# Autodesk Inventor assembly: Square Frame
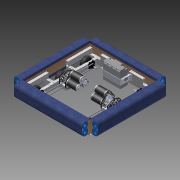
[picture p0: Inventor's stored thumbnail of the model, 180x180]
Saved by Autodesk Inventor 2015 SP1 (Build 190203100, 203)
## iProperties
Created: 2014-12-21
Part Number: Square Frame
Document SubType Name: Assembly
Designer: Jarod
Author: Jarod
## Documents named in this file (23)
- C:\Users\Jarod\Documents\Westview\Robotics\FRC\2015\CAD\Ideas\Square Frame\Square Frame.iam
- C:\Users\Jarod\Documents\Westview\Robotics\FRC\2015\CAD\Ideas\Square Frame\Square Frame Parts\frame_wide.ipt
- C:\Users\Jarod\Documents\Westview\Robotics\FRC\2015\CAD\Ideas\Square Frame\Square Frame Parts\frame_long.ipt
- C:\Users\Jarod\Documents\Westview\Robotics\FRC\2015\CAD\Ideas\Square Frame\Square Frame Parts\Imported Components\Versablock (217-3432)\Versablock (217-3432).ipt
- C:\Users\Jarod\Documents\Westview\Robotics\FRC\2015\CAD\Ideas\Square Frame\Square Frame Parts\Imported Components\0.5 hex bearing (217-2734)\0.5 hex bearing (217-2734).ipt
- C:\Users\Jarod\Documents\Westview\Robotics\FRC\2015\CAD\Ideas\Square Frame\Square Frame Parts\Imported Components\VersaFrame Gusset (217-3557)\VersaFrame Gusset (217-3557).ipt
- C:\Users\Jarod\Documents\Westview\Robotics\FRC\2015\CAD\Ideas\Square Frame\Square Frame Parts\Imported Components\Colson Wheel (4 x 1.5, 0.5 Hex bore) (217-4052)\Colson Wheel (4 x 1.5, 0.5 Hex bore) (217-4052).ipt
- C:\Users\Jarod\Documents\Westview\Robotics\FRC\2015\CAD\Ideas\Square Frame\Square Frame Parts\Imported Components\WCP Single Speed, Double Reduction Gearbox, West Coast Version (217-3422)\WCP Single Speed, Doub.iam
- C:\Users\Jarod\Documents\Westview\Robotics\FRC\2015\CAD\Ideas\Square Frame\Square Frame Parts\Imported Components\0.5 hex hub #35 sprocket 15t double (217-2656)\0.5 hex hub #35 sprocket 15t double (217-2656).ipt
- C:\Users\Jarod\Documents\Westview\Robotics\FRC\2015\CAD\Ideas\Square Frame\Square Frame Parts\Imported Components\0.5 hex hub #35 sprocket 15t (217-2660)\0.5 hex hub #35 sprocket 15t (217-2660).ipt
- C:\Users\Jarod\Documents\Westview\Robotics\FRC\2015\CAD\Ideas\Square Frame\Square Frame Parts\axle.ipt
- C:\Users\Jarod\Documents\Westview\Robotics\FRC\2015\CAD\Ideas\Square Frame\Square Frame Parts\Imported Components\0.5 hex collar (217-2737)\0.5 hex collar (217-2737).ipt
- C:\Users\Jarod\Documents\Westview\Robotics\FRC\2015\CAD\Ideas\Square Frame\Square Frame Parts\Imported Components\WCP Single Speed, Double Reduction Gearbox, West Coast Version (217-3422)\217-2758-001 Rev1.ipt
- C:\Users\Jarod\Documents\Westview\Robotics\FRC\2015\CAD\Ideas\Square Frame\Square Frame Parts\Imported Components\WCP Cam (217-3431)\WCP Cam (217-3431).ipt
- C:\Users\Jarod\Documents\Westview\Robotics\FRC\2015\CAD\Ideas\Square Frame\Square Frame Parts\base.ipt
- C:\Users\Jarod\Documents\Westview\Robotics\FRC\2015\CAD\Ideas\Square Frame\Square Frame Parts\frame_side.ipt
- C:\Users\Jarod\Documents\Westview\Robotics\FRC\2015\CAD\Ideas\Square Frame\Square Frame Parts\frame_side_bumper.ipt
- C:\Users\Jarod\Documents\Westview\Robotics\FRC\2015\CAD\Ideas\Square Frame\Square Frame Parts\bumper.iam
- C:\Users\Jarod\Documents\Westview\Robotics\FRC\2015\CAD\Ideas\Square Frame\Square Frame Parts\frame_front_bumper.ipt
- C:\Users\Jarod\Documents\Westview\Robotics\FRC\2015\CAD\Ideas\Square Frame\Square Frame Parts\chain (71 links).ipt
- C:\Users\Jarod\Documents\Westview\Robotics\FRC\2015\CAD\Ideas\Square Frame\Square Frame Parts\Imported Components\VersaFrame Gusset (217-3557)\VersaFrame Gusset (217-3557) (modified).ipt
- C:\Users\Jarod\Documents\Westview\Robotics\FRC\2015\CAD\Ideas\Square Frame\Square Frame Parts\battery.ipt
- C:\Users\Jarod\Documents\Westview\Robotics\FRC\2015\CAD\Ideas\Square Frame\Square Frame Parts\Imported Components\Battery Tray\Battery Tray_TOP.iam
## Components (95 placed, 22 different names)
1. frame_wide:1 — Flush:1, Flush:2, Flush:3, Mate:1, Mate:2, Mate:28, Mate:29, Mate:38, Mate:39, Mate:52, Mate:53, Flush:13, Flush:14, Mate:56, Mate:57, Flush:23, Flush:24, Flush:37, Flush:63, Flush:64, Mate:186, Flush:65, Flush:66, Mate:188, Flush:69, Flush:70, Mate:190, Flush:75, Flush:76, Mate:192, Mate:194, Flush:77, Mate:198, Flush:79, Mate:204, Flush:82, Mate:235, Mate:236
2. frame_wide:2 — Flush:3, Mate:3, Mate:32, Mate:33, Mate:34, Mate:35, Mate:54, Mate:55, Flush:17, Flush:18, Mate:58, Mate:59, Flush:25, Flush:26, Flush:63, Mate:187, Mate:189, Flush:71, Flush:72, Flush:73, Flush:74, Mate:195, Flush:78, Mate:200, Flush:80, Mate:202, Flush:81, Mate:232, Mate:233, Mate:234, Mate:237, Mate:238
3. frame_long:1 — Flush:1, Mate:2, Mate:3, Mate:4, Mate:5, Mate:8, Mate:9, Mate:16, Mate:17, Mate:20, Mate:21, Flush:15, Flush:16, Flush:19, Flush:20, Mate:60, Mate:61, Mate:64, Mate:65, Mate:72, Mate:73, Mate:74, Mate:161, Mate:162, Cylindrical:15, Cylindrical:16, Flush:38, Flush:39, Flush:40, Mate:166, Mate:167, Mate:181, Flush:64, Mate:208, Mate:209, Mate:210, Mate:211, Mate:220, Flush:83, Mate:221, Flush:84, Mate:222, Flush:85, Mate:223, Flush:86, Mate:228, Mate:229
4. frame_long:2 — Flush:2, Mate:1, Mate:10, Mate:11, Mate:14, Mate:15, Mate:22, Mate:23, Mate:26, Mate:27, Flush:21, Flush:22, Flush:27, Flush:28, Mate:66, Mate:67, Mate:70, Mate:71, Mate:75, Mate:76, Mate:77, Mate:159, Mate:160, Cylindrical:13, Cylindrical:14, Flush:41, Flush:42, Mate:181, Mate:184, Mate:185, Mate:212, Mate:213, Mate:214, Mate:215, Mate:224, Flush:87, Mate:225, Flush:88, Mate:226, Flush:89, Mate:227, Flush:90, Mate:230, Mate:231
5. frame_side:1 — Flush:39, Mate:166, Flush:91, Flush:92
6. frame_side:2 — Flush:40, Mate:167, Flush:93, Flush:94
7. frame_side:3 — Flush:41, Mate:184, Flush:95, Flush:96
8. frame_side:4 — Flush:42, Mate:185, Flush:97, Flush:98
9. frame_side_bumper:1 — Mate:186, Flush:65, Flush:66, Mate:196
10. frame_side_bumper:2 — Mate:187, Flush:71, Flush:72
11. frame_side_bumper:3 — Mate:188, Flush:69, Flush:70, Mate:197
12. frame_side_bumper:4 — Mate:189, Flush:73, Flush:74
13. frame_front_bumper:1 — Mate:198, Flush:79, Mate:236, Mate:239
14. frame_front_bumper:2 — Mate:200, Flush:80, Mate:238, Mate:240
15. frame_front_bumper:3 — Mate:204, Flush:82, Mate:235
16. frame_front_bumper:4 — Mate:202, Flush:81, Mate:237
17. base:1 — Mate:163, Flush:37, Flush:38
18. VersaFrame Gusset (217-3557):1 — Mate:52, Flush:13, Flush:15
19. VersaFrame Gusset (217-3557):2 — Mate:53, Flush:14, Flush:16, Mate:163
20. VersaFrame Gusset (217-3557):3 — Mate:54, Flush:17, Flush:20
21. VersaFrame Gusset (217-3557):4 — Mate:55, Flush:18, Flush:19
22. VersaFrame Gusset (217-3557):5 — Mate:57, Flush:22, Flush:23
23. VersaFrame Gusset (217-3557):6 — Mate:56, Flush:21, Flush:24
24. VersaFrame Gusset (217-3557):7 — Mate:58, Flush:25, Flush:28
25. VersaFrame Gusset (217-3557):8 — Mate:59, Flush:26, Flush:27
26. VersaFrame Gusset (217-3557) (modified):1 — Mate:220, Flush:83, Flush:91, Mate:228
27. VersaFrame Gusset (217-3557) (modified):2 — Mate:221, Flush:84, Flush:92
28. VersaFrame Gusset (217-3557) (modified):3 — Mate:222, Flush:85, Flush:93, Mate:229
29. VersaFrame Gusset (217-3557) (modified):4 — Mate:223, Flush:86, Flush:94
30. VersaFrame Gusset (217-3557) (modified):5 — Mate:224, Flush:87, Flush:95, Mate:230
31. VersaFrame Gusset (217-3557) (modified):6 — Mate:225, Flush:88, Flush:96
32. VersaFrame Gusset (217-3557) (modified):7 — Mate:226, Flush:89, Flush:97, Mate:231
33. VersaFrame Gusset (217-3557) (modified):8 — Mate:227, Flush:90, Flush:98
34. bumper:1 [sub-assembly] — Mate:190, Flush:75, Mate:196
35. bumper:2 [sub-assembly] — Flush:76, Mate:192, Mate:197
36. bumper:3 [sub-assembly] — Mate:194, Flush:77, Mate:239
37. bumper:4 [sub-assembly] — Mate:195, Flush:78, Mate:240
38. WCP Single Speed, Doub:1 [sub-assembly] — Mate:72, Mate:73, Mate:74, Mate:81, Mate:82, Mate:83, Mate:90, Mate:91, Mate:128, Mate:129, Mate:130
39. WCP Single Speed, Doub:2 [sub-assembly] — Mate:75, Mate:76, Mate:77, Mate:78, Mate:79, Mate:80, Mate:104, Mate:105, Mate:148, Mate:149, Mate:150
40. Versablock (217-3432):1 — Mate:4, Mate:17, Mate:38, Cylindrical:2
41. Versablock (217-3432):2 — Mate:5, Mate:16, Mate:39, Cylindrical:1
42. Versablock (217-3432):5 — Mate:9, Mate:21, Mate:34, Cylindrical:5
43. Versablock (217-3432):6 — Mate:8, Mate:20, Mate:35, Cylindrical:6
44. Versablock (217-3432):7 — Mate:10, Mate:22, Mate:28, Cylindrical:7
45. Versablock (217-3432):8 — Mate:11, Mate:23, Mate:29, Cylindrical:8
46. Versablock (217-3432):11 — Mate:14, Mate:27, Mate:32, Cylindrical:11
47. Versablock (217-3432):12 — Mate:15, Mate:26, Mate:33, Cylindrical:12
48. axle:1 — Mate:84, Mate:85, Mate:86, Mate:87, Mate:88, Mate:89, Mate:118, Mate:119, Mate:120, Mate:121, Mate:122, Mate:123, Flush:33
49. axle:2 — Mate:92, Mate:93, Mate:94, Mate:95, Mate:96, Mate:97, Mate:114, Mate:115, Mate:132, Mate:133, Mate:134, Mate:135, Flush:34
50. axle:3 — Mate:98, Mate:99, Mate:100, Mate:101, Mate:102, Mate:103, Mate:138, Mate:139, Mate:140, Mate:141, Mate:142, Mate:143, Flush:35
51. axle:4 — Mate:106, Mate:107, Mate:108, Mate:109, Mate:110, Mate:111, Mate:112, Mate:113, Mate:152, Mate:153, Mate:156, Mate:157, Flush:36
52. 0.5 hex bearing (217-2734):1 — Mate:60, Cylindrical:1, Mate:88, Mate:89, Mate:126
53. 0.5 hex bearing (217-2734):2 — Mate:61, Cylindrical:2
54. 0.5 hex bearing (217-2734):5 — Mate:64, Cylindrical:6, Mate:96, Mate:97, Mate:180
55. 0.5 hex bearing (217-2734):6 — Mate:65, Cylindrical:5, Mate:116
56. 0.5 hex bearing (217-2734):7 — Mate:66, Cylindrical:8, Mate:102, Mate:103, Mate:146
57. 0.5 hex bearing (217-2734):8 — Mate:67, Cylindrical:7
58. 0.5 hex bearing (217-2734):11 — Mate:70, Cylindrical:12, Mate:110, Mate:111, Mate:155
59. 0.5 hex bearing (217-2734):12 — Mate:71, Cylindrical:11, Mate:117
60. Colson Wheel (4 x 1.5, 0.5 Hex bore) (217-4052):2 — Mate:90, Mate:91, Mate:128, Mate:131
61. Colson Wheel (4 x 1.5, 0.5 Hex bore) (217-4052):3 — Mate:92, Mate:93, Mate:136, Mate:180
62. Colson Wheel (4 x 1.5, 0.5 Hex bore) (217-4052):4 — Mate:98, Mate:99, Mate:146, Mate:147
63. Colson Wheel (4 x 1.5, 0.5 Hex bore) (217-4052):5 — Mate:104, Mate:105, Mate:148, Mate:151
64. Colson Wheel (4 x 1.5, 0.5 Hex bore) (217-4052):6 — Mate:106, Mate:107, Mate:155, Mate:158
65. Colson Wheel (4 x 1.5, 0.5 Hex bore) (217-4052):1 — Mate:84, Mate:85, Mate:126, Mate:127
66. 0.5 hex hub #35 sprocket 15t double (217-2656):1 — Mate:78, Mate:79, Mate:80, Flush:31, Flush:32
67. 0.5 hex hub #35 sprocket 15t double (217-2656):2 — Mate:81, Mate:82, Mate:83, Flush:29, Flush:30
68. 0.5 hex hub #35 sprocket 15t (217-2660):1 — Flush:32, Mate:108, Mate:109, Mate:154, Mate:217
69. 0.5 hex hub #35 sprocket 15t (217-2660):2 — Flush:29, Mate:94, Mate:95, Mate:137, Mate:218
70. 0.5 hex hub #35 sprocket 15t (217-2660):3 — Flush:30, Mate:86, Mate:87, Mate:124, Mate:125, Mate:219
71. 0.5 hex hub #35 sprocket 15t (217-2660):4 — Flush:31, Mate:100, Mate:101, Mate:144, Mate:145, Mate:216
72. 217-2758-001 Rev1:1 — Mate:112, Mate:113, Mate:117
73. 217-2758-001 Rev1:2 — Mate:114, Mate:115, Mate:116
74. 0.5 hex collar (217-2737):1 — Mate:118, Mate:119, Mate:127, Flush:33
75. 0.5 hex collar (217-2737):2 — Mate:120, Mate:121, Mate:125
76. 0.5 hex collar (217-2737):3 — Mate:122, Mate:123, Mate:124
77. 0.5 hex collar (217-2737):4 — Mate:129, Mate:130, Mate:131
78. 0.5 hex collar (217-2737):5 — Mate:134, Mate:135, Mate:136, Flush:34
79. 0.5 hex collar (217-2737):6 — Mate:132, Mate:133, Mate:137
80. 0.5 hex collar (217-2737):7 — Mate:142, Mate:143, Mate:147, Flush:35
81. 0.5 hex collar (217-2737):8 — Mate:140, Mate:141, Mate:145
82. 0.5 hex collar (217-2737):9 — Mate:138, Mate:139, Mate:144
83. 0.5 hex collar (217-2737):10 — Mate:149, Mate:150, Mate:151
84. 0.5 hex collar (217-2737):11 — Mate:156, Mate:157, Mate:158, Flush:36
85. 0.5 hex collar (217-2737):12 — Mate:152, Mate:153, Mate:154
86. chain (71 links):1 — Mate:208, Mate:209, Mate:219
87. chain (71 links):2 — Mate:210, Mate:211, Mate:218
88. chain (71 links):3 — Mate:212, Mate:213, Mate:216
89. chain (71 links):4 — Mate:214, Mate:215, Mate:217
90. WCP Cam (217-3431):1 — Mate:162, Cylindrical:16
91. WCP Cam (217-3431):2 — Mate:161, Cylindrical:15
92. WCP Cam (217-3431):3 — Mate:160, Cylindrical:14
93. WCP Cam (217-3431):4 — Mate:159, Cylindrical:13
94. battery:1
95. Battery Tray_TOP:1 [sub-assembly] — Mate:232, Mate:233, Mate:234
## Relationships (267: Mate 188, Flush 67, CylindricalJoint 12)
- Flush:1: frame_wide:1 ↔ frame_long:1
- Flush:2: frame_wide:1 ↔ frame_long:2
- Flush:3: frame_wide:1 ↔ frame_wide:2
- Mate:1: frame_wide:1 ↔ frame_long:2
- Mate:2: frame_wide:1 ↔ frame_long:1
- Mate:3: frame_wide:2 ↔ frame_long:1
- Mate:4: frame_long:1 ↔ Versablock (217-3432):1
- Mate:5: frame_long:1 ↔ Versablock (217-3432):2
- Mate:8: frame_long:1 ↔ Versablock (217-3432):6
- Mate:9: frame_long:1 ↔ Versablock (217-3432):5
- Mate:10: frame_long:2 ↔ Versablock (217-3432):7
- Mate:11: frame_long:2 ↔ Versablock (217-3432):8
- Mate:14: frame_long:2 ↔ Versablock (217-3432):11
- Mate:15: frame_long:2 ↔ Versablock (217-3432):12
- Mate:16: frame_long:1 ↔ Versablock (217-3432):2
- Mate:17: frame_long:1 ↔ Versablock (217-3432):1
- Mate:20: frame_long:1 ↔ Versablock (217-3432):6
- Mate:21: frame_long:1 ↔ Versablock (217-3432):5
- Mate:22: frame_long:2 ↔ Versablock (217-3432):7
- Mate:23: frame_long:2 ↔ Versablock (217-3432):8
- Mate:26: frame_long:2 ↔ Versablock (217-3432):12
- Mate:27: frame_long:2 ↔ Versablock (217-3432):11
- Mate:28 (63.5 mm): frame_wide:1 ↔ Versablock (217-3432):7
- Mate:29 (63.5 mm): frame_wide:1 ↔ Versablock (217-3432):8
- Mate:32 (63.5 mm): frame_wide:2 ↔ Versablock (217-3432):11
- Mate:33 (63.5 mm): frame_wide:2 ↔ Versablock (217-3432):12
- Mate:34 (63.5 mm): frame_wide:2 ↔ Versablock (217-3432):5
- Mate:35 (63.5 mm): frame_wide:2 ↔ Versablock (217-3432):6
- Mate:38 (63.5 mm): frame_wide:1 ↔ Versablock (217-3432):1
- Mate:39 (63.5 mm): frame_wide:1 ↔ Versablock (217-3432):2
- Mate:52: frame_wide:1 ↔ VersaFrame Gusset (217-3557):1
- Mate:53: frame_wide:1 ↔ VersaFrame Gusset (217-3557):2
- Flush:13: frame_wide:1 ↔ VersaFrame Gusset (217-3557):1
- Flush:14: frame_wide:1 ↔ VersaFrame Gusset (217-3557):2
- Flush:15: frame_long:1 ↔ VersaFrame Gusset (217-3557):1
- Flush:16: frame_long:1 ↔ VersaFrame Gusset (217-3557):2
- Mate:54: frame_wide:2 ↔ VersaFrame Gusset (217-3557):3
- Mate:55: frame_wide:2 ↔ VersaFrame Gusset (217-3557):4
- Flush:17: frame_wide:2 ↔ VersaFrame Gusset (217-3557):3
- Flush:18: frame_wide:2 ↔ VersaFrame Gusset (217-3557):4
- Flush:19: frame_long:1 ↔ VersaFrame Gusset (217-3557):4
- Flush:20: frame_long:1 ↔ VersaFrame Gusset (217-3557):3
- Mate:56: frame_wide:1 ↔ VersaFrame Gusset (217-3557):6
- Mate:57: frame_wide:1 ↔ VersaFrame Gusset (217-3557):5
- Flush:21: frame_long:2 ↔ VersaFrame Gusset (217-3557):6
- Flush:22: frame_long:2 ↔ VersaFrame Gusset (217-3557):5
- Flush:23: frame_wide:1 ↔ VersaFrame Gusset (217-3557):5
- Flush:24: frame_wide:1 ↔ VersaFrame Gusset (217-3557):6
- Mate:58: frame_wide:2 ↔ VersaFrame Gusset (217-3557):7
- Mate:59: frame_wide:2 ↔ VersaFrame Gusset (217-3557):8
- Flush:25: frame_wide:2 ↔ VersaFrame Gusset (217-3557):7
- Flush:26: frame_wide:2 ↔ VersaFrame Gusset (217-3557):8
- Flush:27: frame_long:2 ↔ VersaFrame Gusset (217-3557):8
- Flush:28: frame_long:2 ↔ VersaFrame Gusset (217-3557):7
- Mate:60: frame_long:1 ↔ 0.5 hex bearing (217-2734):1
- Cylindrical:1: Versablock (217-3432):2 ↔ 0.5 hex bearing (217-2734):1
- Mate:61: frame_long:1 ↔ 0.5 hex bearing (217-2734):2
- Cylindrical:2: Versablock (217-3432):1 ↔ 0.5 hex bearing (217-2734):2
- Mate:64: frame_long:1 ↔ 0.5 hex bearing (217-2734):5
- Mate:65: frame_long:1 ↔ 0.5 hex bearing (217-2734):6
- Cylindrical:5: Versablock (217-3432):5 ↔ 0.5 hex bearing (217-2734):6
- Cylindrical:6: Versablock (217-3432):6 ↔ 0.5 hex bearing (217-2734):5
- Mate:66: frame_long:2 ↔ 0.5 hex bearing (217-2734):7
- Mate:67: frame_long:2 ↔ 0.5 hex bearing (217-2734):8
- Cylindrical:7: Versablock (217-3432):7 ↔ 0.5 hex bearing (217-2734):8
- Cylindrical:8: Versablock (217-3432):8 ↔ 0.5 hex bearing (217-2734):7
- Mate:70: frame_long:2 ↔ 0.5 hex bearing (217-2734):11
- Mate:71: frame_long:2 ↔ 0.5 hex bearing (217-2734):12
- Cylindrical:11: Versablock (217-3432):11 ↔ 0.5 hex bearing (217-2734):12
- Cylindrical:12: Versablock (217-3432):12 ↔ 0.5 hex bearing (217-2734):11
- Mate:72: frame_long:1 ↔ WCP Single Speed, Doub:1
- Mate:73: frame_long:1 ↔ WCP Single Speed, Doub:1
- Mate:74: frame_long:1 ↔ WCP Single Speed, Doub:1
- Mate:75: frame_long:2 ↔ WCP Single Speed, Doub:2
- Mate:76: frame_long:2 ↔ WCP Single Speed, Doub:2
- Mate:77: frame_long:2 ↔ WCP Single Speed, Doub:2
- Mate:78: WCP Single Speed, Doub:2 ↔ 0.5 hex hub #35 sprocket 15t double (217-2656):1
- Mate:79: WCP Single Speed, Doub:2 ↔ 0.5 hex hub #35 sprocket 15t double (217-2656):1
- Mate:80: WCP Single Speed, Doub:2 ↔ 0.5 hex hub #35 sprocket 15t double (217-2656):1
- Mate:81: WCP Single Speed, Doub:1 ↔ 0.5 hex hub #35 sprocket 15t double (217-2656):2
- Mate:82: WCP Single Speed, Doub:1 ↔ 0.5 hex hub #35 sprocket 15t double (217-2656):2
- Mate:83: WCP Single Speed, Doub:1 ↔ 0.5 hex hub #35 sprocket 15t double (217-2656):2
- Flush:29: 0.5 hex hub #35 sprocket 15t double (217-2656):2 ↔ 0.5 hex hub #35 sprocket 15t (217-2660):2
- Flush:30: 0.5 hex hub #35 sprocket 15t double (217-2656):2 ↔ 0.5 hex hub #35 sprocket 15t (217-2660):3
- Flush:31: 0.5 hex hub #35 sprocket 15t double (217-2656):1 ↔ 0.5 hex hub #35 sprocket 15t (217-2660):4
- Flush:32: 0.5 hex hub #35 sprocket 15t double (217-2656):1 ↔ 0.5 hex hub #35 sprocket 15t (217-2660):1
- Mate:84: axle:1 ↔ Colson Wheel (4 x 1.5, 0.5 Hex bore) (217-4052):1
- Mate:85: axle:1 ↔ Colson Wheel (4 x 1.5, 0.5 Hex bore) (217-4052):1
- Mate:86: axle:1 ↔ 0.5 hex hub #35 sprocket 15t (217-2660):3
- Mate:87: axle:1 ↔ 0.5 hex hub #35 sprocket 15t (217-2660):3
- Mate:88: axle:1 ↔ 0.5 hex bearing (217-2734):1
- Mate:89: axle:1 ↔ 0.5 hex bearing (217-2734):1
- Mate:90: WCP Single Speed, Doub:1 ↔ Colson Wheel (4 x 1.5, 0.5 Hex bore) (217-4052):2
- Mate:91: WCP Single Speed, Doub:1 ↔ Colson Wheel (4 x 1.5, 0.5 Hex bore) (217-4052):2
- Mate:92: axle:2 ↔ Colson Wheel (4 x 1.5, 0.5 Hex bore) (217-4052):3
- Mate:93: axle:2 ↔ Colson Wheel (4 x 1.5, 0.5 Hex bore) (217-4052):3
- Mate:94: axle:2 ↔ 0.5 hex hub #35 sprocket 15t (217-2660):2
- Mate:95: axle:2 ↔ 0.5 hex hub #35 sprocket 15t (217-2660):2
- Mate:96: axle:2 ↔ 0.5 hex bearing (217-2734):5
- Mate:97: axle:2 ↔ 0.5 hex bearing (217-2734):5
- Mate:98: axle:3 ↔ Colson Wheel (4 x 1.5, 0.5 Hex bore) (217-4052):4
- Mate:99: axle:3 ↔ Colson Wheel (4 x 1.5, 0.5 Hex bore) (217-4052):4
- Mate:100: axle:3 ↔ 0.5 hex hub #35 sprocket 15t (217-2660):4
- Mate:101: axle:3 ↔ 0.5 hex hub #35 sprocket 15t (217-2660):4
- Mate:102: axle:3 ↔ 0.5 hex bearing (217-2734):7
- Mate:103: axle:3 ↔ 0.5 hex bearing (217-2734):7
- Mate:104: WCP Single Speed, Doub:2 ↔ Colson Wheel (4 x 1.5, 0.5 Hex bore) (217-4052):5
- Mate:105: WCP Single Speed, Doub:2 ↔ Colson Wheel (4 x 1.5, 0.5 Hex bore) (217-4052):5
- Mate:106: axle:4 ↔ Colson Wheel (4 x 1.5, 0.5 Hex bore) (217-4052):6
- Mate:107: axle:4 ↔ Colson Wheel (4 x 1.5, 0.5 Hex bore) (217-4052):6
- Mate:108: axle:4 ↔ 0.5 hex hub #35 sprocket 15t (217-2660):1
- Mate:109: axle:4 ↔ 0.5 hex hub #35 sprocket 15t (217-2660):1
- Mate:110: axle:4 ↔ 0.5 hex bearing (217-2734):11
- Mate:111: axle:4 ↔ 0.5 hex bearing (217-2734):11
- Mate:112: axle:4 ↔ 217-2758-001 Rev1:1
- Mate:113: axle:4 ↔ 217-2758-001 Rev1:1
- Mate:114: axle:2 ↔ 217-2758-001 Rev1:2
- Mate:115: axle:2 ↔ 217-2758-001 Rev1:2
- Mate:116: 0.5 hex bearing (217-2734):6 ↔ 217-2758-001 Rev1:2
- Mate:117: 0.5 hex bearing (217-2734):12 ↔ 217-2758-001 Rev1:1
- Mate:118: axle:1 ↔ 0.5 hex collar (217-2737):1
- Mate:119: axle:1 ↔ 0.5 hex collar (217-2737):1
- Mate:120: axle:1 ↔ 0.5 hex collar (217-2737):2
- Mate:121: axle:1 ↔ 0.5 hex collar (217-2737):2
- Mate:122: axle:1 ↔ 0.5 hex collar (217-2737):3
- Mate:123: axle:1 ↔ 0.5 hex collar (217-2737):3
- Mate:124: 0.5 hex hub #35 sprocket 15t (217-2660):3 ↔ 0.5 hex collar (217-2737):3
- Mate:125: 0.5 hex hub #35 sprocket 15t (217-2660):3 ↔ 0.5 hex collar (217-2737):2
- Mate:126: 0.5 hex bearing (217-2734):1 ↔ Colson Wheel (4 x 1.5, 0.5 Hex bore) (217-4052):1
- Mate:127: Colson Wheel (4 x 1.5, 0.5 Hex bore) (217-4052):1 ↔ 0.5 hex collar (217-2737):1
- Flush:33 (-12.7 mm): axle:1 ↔ 0.5 hex collar (217-2737):1
- Mate:128: WCP Single Speed, Doub:1 ↔ Colson Wheel (4 x 1.5, 0.5 Hex bore) (217-4052):2
- Mate:129: WCP Single Speed, Doub:1 ↔ 0.5 hex collar (217-2737):4
- Mate:130: WCP Single Speed, Doub:1 ↔ 0.5 hex collar (217-2737):4
- Mate:131: Colson Wheel (4 x 1.5, 0.5 Hex bore) (217-4052):2 ↔ 0.5 hex collar (217-2737):4
- Mate:132: axle:2 ↔ 0.5 hex collar (217-2737):6
- Mate:133: axle:2 ↔ 0.5 hex collar (217-2737):6
- Mate:134: axle:2 ↔ 0.5 hex collar (217-2737):5
- Mate:135: axle:2 ↔ 0.5 hex collar (217-2737):5
- Mate:136: Colson Wheel (4 x 1.5, 0.5 Hex bore) (217-4052):3 ↔ 0.5 hex collar (217-2737):5
- Mate:137: 0.5 hex hub #35 sprocket 15t (217-2660):2 ↔ 0.5 hex collar (217-2737):6
- Flush:34 (-12.7 mm): axle:2 ↔ 0.5 hex collar (217-2737):5
- Mate:138: axle:3 ↔ 0.5 hex collar (217-2737):9
- Mate:139: axle:3 ↔ 0.5 hex collar (217-2737):9
- Mate:140: axle:3 ↔ 0.5 hex collar (217-2737):8
- Mate:141: axle:3 ↔ 0.5 hex collar (217-2737):8
- Mate:142: axle:3 ↔ 0.5 hex collar (217-2737):7
- Mate:143: axle:3 ↔ 0.5 hex collar (217-2737):7
- Mate:144: 0.5 hex hub #35 sprocket 15t (217-2660):4 ↔ 0.5 hex collar (217-2737):9
- Mate:145: 0.5 hex hub #35 sprocket 15t (217-2660):4 ↔ 0.5 hex collar (217-2737):8
- Mate:146: 0.5 hex bearing (217-2734):7 ↔ Colson Wheel (4 x 1.5, 0.5 Hex bore) (217-4052):4
- Mate:147: Colson Wheel (4 x 1.5, 0.5 Hex bore) (217-4052):4 ↔ 0.5 hex collar (217-2737):7
- Flush:35 (-12.7 mm): axle:3 ↔ 0.5 hex collar (217-2737):7
- Mate:148: WCP Single Speed, Doub:2 ↔ Colson Wheel (4 x 1.5, 0.5 Hex bore) (217-4052):5
- Mate:149: WCP Single Speed, Doub:2 ↔ 0.5 hex collar (217-2737):10
- Mate:150: WCP Single Speed, Doub:2 ↔ 0.5 hex collar (217-2737):10
- Mate:151: Colson Wheel (4 x 1.5, 0.5 Hex bore) (217-4052):5 ↔ 0.5 hex collar (217-2737):10
- Mate:152: axle:4 ↔ 0.5 hex collar (217-2737):12
- Mate:153: axle:4 ↔ 0.5 hex collar (217-2737):12
- Mate:154: 0.5 hex hub #35 sprocket 15t (217-2660):1 ↔ 0.5 hex collar (217-2737):12
- Mate:155: 0.5 hex bearing (217-2734):11 ↔ Colson Wheel (4 x 1.5, 0.5 Hex bore) (217-4052):6
- Mate:156: axle:4 ↔ 0.5 hex collar (217-2737):11
- Mate:157: axle:4 ↔ 0.5 hex collar (217-2737):11
- Mate:158: Colson Wheel (4 x 1.5, 0.5 Hex bore) (217-4052):6 ↔ 0.5 hex collar (217-2737):11
- Flush:36 (-12.7 mm): axle:4 ↔ 0.5 hex collar (217-2737):11
- Mate:159: frame_long:2 ↔ WCP Cam (217-3431):4
- Mate:160: frame_long:2 ↔ WCP Cam (217-3431):3
- Mate:161: frame_long:1 ↔ WCP Cam (217-3431):2
- Mate:162: frame_long:1 ↔ WCP Cam (217-3431):1
- Cylindrical:13: frame_long:2 ↔ WCP Cam (217-3431):4
- Cylindrical:14: frame_long:2 ↔ WCP Cam (217-3431):3
- Cylindrical:15: frame_long:1 ↔ WCP Cam (217-3431):2
- Cylindrical:16: frame_long:1 ↔ WCP Cam (217-3431):1
- Mate:163: base:1 ↔ VersaFrame Gusset (217-3557):2
- Flush:37: frame_wide:1 ↔ base:1
- Flush:38: frame_long:1 ↔ base:1
- Flush:39: frame_long:1 ↔ frame_side:1
- Flush:40: frame_long:1 ↔ frame_side:2
- Flush:41: frame_long:2 ↔ frame_side:3
- Flush:42: frame_long:2 ↔ frame_side:4
- Mate:166: frame_long:1 ↔ frame_side:1
- Mate:167: frame_long:1 ↔ frame_side:2
- Mate:180: 0.5 hex bearing (217-2734):5 ↔ Colson Wheel (4 x 1.5, 0.5 Hex bore) (217-4052):3
- Mate:181 (508 mm): frame_long:1 ↔ frame_long:2
- Mate:184: frame_long:2 ↔ frame_side:3
- Mate:185: frame_long:2 ↔ frame_side:4
- Flush:63: frame_wide:1 ↔ frame_wide:2
- Flush:64 (76.2 mm): frame_wide:1 ↔ frame_long:1
- Mate:186: frame_wide:1 ↔ frame_side_bumper:1
- Flush:65: frame_wide:1 ↔ frame_side_bumper:1
- Flush:66: frame_wide:1 ↔ frame_side_bumper:1
- Mate:187: frame_wide:2 ↔ frame_side_bumper:2
- Mate:188: frame_wide:1 ↔ frame_side_bumper:3
- Flush:69: frame_wide:1 ↔ frame_side_bumper:3
- Flush:70: frame_wide:1 ↔ frame_side_bumper:3
- Mate:189: frame_wide:2 ↔ frame_side_bumper:4
- Flush:71: frame_wide:2 ↔ frame_side_bumper:2
- Flush:72: frame_wide:2 ↔ frame_side_bumper:2
- Flush:73: frame_wide:2 ↔ frame_side_bumper:4
- Flush:74: frame_wide:2 ↔ frame_side_bumper:4
- Mate:190: frame_wide:1 ↔ bumper:1
- Flush:75: frame_wide:1 ↔ bumper:1
- Flush:76: frame_wide:1 ↔ bumper:2
- Mate:192: frame_wide:1 ↔ bumper:2
- Mate:194: frame_wide:1 ↔ bumper:3
- Flush:77: frame_wide:1 ↔ bumper:3
- Mate:195: frame_wide:2 ↔ bumper:4
- Flush:78: frame_wide:2 ↔ bumper:4
- Mate:196: frame_side_bumper:1 ↔ bumper:1
- Mate:197: frame_side_bumper:3 ↔ bumper:2
- Mate:198: frame_wide:1 ↔ frame_front_bumper:1
- Flush:79: frame_wide:1 ↔ frame_front_bumper:1
- Mate:200: frame_wide:2 ↔ frame_front_bumper:2
- Flush:80: frame_wide:2 ↔ frame_front_bumper:2
- Mate:202: frame_wide:2 ↔ frame_front_bumper:4
- Flush:81: frame_wide:2 ↔ frame_front_bumper:4
- Mate:204: frame_wide:1 ↔ frame_front_bumper:3
- Flush:82: frame_wide:1 ↔ frame_front_bumper:3
- Mate:208: frame_long:1 ↔ chain (71 links):1
- Mate:209: frame_long:1 ↔ chain (71 links):1
- Mate:210: frame_long:1 ↔ chain (71 links):2
- Mate:211: frame_long:1 ↔ chain (71 links):2
- Mate:212: frame_long:2 ↔ chain (71 links):3
- Mate:213: frame_long:2 ↔ chain (71 links):3
- Mate:214: frame_long:2 ↔ chain (71 links):4
- Mate:215: frame_long:2 ↔ chain (71 links):4
- Mate:216: 0.5 hex hub #35 sprocket 15t (217-2660):4 ↔ chain (71 links):3
- Mate:217: 0.5 hex hub #35 sprocket 15t (217-2660):1 ↔ chain (71 links):4
- Mate:218: 0.5 hex hub #35 sprocket 15t (217-2660):2 ↔ chain (71 links):2
- Mate:219: 0.5 hex hub #35 sprocket 15t (217-2660):3 ↔ chain (71 links):1
- Mate:220: frame_long:1 ↔ VersaFrame Gusset (217-3557) (modified):1
- Flush:83: frame_long:1 ↔ VersaFrame Gusset (217-3557) (modified):1
- Mate:221: frame_long:1 ↔ VersaFrame Gusset (217-3557) (modified):2
- Flush:84: frame_long:1 ↔ VersaFrame Gusset (217-3557) (modified):2
- Mate:222: frame_long:1 ↔ VersaFrame Gusset (217-3557) (modified):3
- Flush:85: frame_long:1 ↔ VersaFrame Gusset (217-3557) (modified):3
- Mate:223: frame_long:1 ↔ VersaFrame Gusset (217-3557) (modified):4
- Flush:86: frame_long:1 ↔ VersaFrame Gusset (217-3557) (modified):4
- Mate:224: frame_long:2 ↔ VersaFrame Gusset (217-3557) (modified):5
- Flush:87: frame_long:2 ↔ VersaFrame Gusset (217-3557) (modified):5
- Mate:225: frame_long:2 ↔ VersaFrame Gusset (217-3557) (modified):6
- Flush:88: frame_long:2 ↔ VersaFrame Gusset (217-3557) (modified):6
- Mate:226: frame_long:2 ↔ VersaFrame Gusset (217-3557) (modified):7
- Flush:89: frame_long:2 ↔ VersaFrame Gusset (217-3557) (modified):7
- Mate:227: frame_long:2 ↔ VersaFrame Gusset (217-3557) (modified):8
- Flush:90: frame_long:2 ↔ VersaFrame Gusset (217-3557) (modified):8
- Flush:91: frame_side:1 ↔ VersaFrame Gusset (217-3557) (modified):1
- Flush:92: frame_side:1 ↔ VersaFrame Gusset (217-3557) (modified):2
- Mate:228: frame_long:1 ↔ VersaFrame Gusset (217-3557) (modified):1
- Flush:93: frame_side:2 ↔ VersaFrame Gusset (217-3557) (modified):3
- Flush:94: frame_side:2 ↔ VersaFrame Gusset (217-3557) (modified):4
- Mate:229: frame_long:1 ↔ VersaFrame Gusset (217-3557) (modified):3
- Flush:95: frame_side:3 ↔ VersaFrame Gusset (217-3557) (modified):5
- Flush:96: frame_side:3 ↔ VersaFrame Gusset (217-3557) (modified):6
- Mate:230: frame_long:2 ↔ VersaFrame Gusset (217-3557) (modified):5
- Flush:97: frame_side:4 ↔ VersaFrame Gusset (217-3557) (modified):7
- Flush:98: frame_side:4 ↔ VersaFrame Gusset (217-3557) (modified):8
- Mate:231: frame_long:2 ↔ VersaFrame Gusset (217-3557) (modified):7
- Mate:232: frame_wide:2 ↔ Battery Tray_TOP:1
- Mate:233 (-12.7 mm): frame_wide:2 ↔ Battery Tray_TOP:1
- Mate:234 (-12.7 mm): frame_wide:2 ↔ Battery Tray_TOP:1
- Mate:235: frame_wide:1 ↔ frame_front_bumper:3
- Mate:236: frame_wide:1 ↔ frame_front_bumper:1
- Mate:237: frame_wide:2 ↔ frame_front_bumper:4
- Mate:238: frame_wide:2 ↔ frame_front_bumper:2
- Mate:239: frame_front_bumper:1 ↔ bumper:3
- Mate:240: frame_front_bumper:2 ↔ bumper:4
